# Autodesk Inventor assembly: hph_002
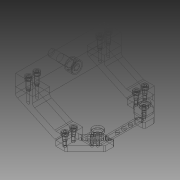
[picture p0: Inventor's stored thumbnail of the model, 180x180]
Saved by Autodesk Inventor 2014 (Build 180170000, 170)
## iProperties
Created: 2014-03-27
Part Number: hph_002
Document SubType Name: Assembly
Designer: stephenholtz
Author: stephenholtz
## Documents named in this file (11)
- C:\Users\stephenholtz\Dropbox\grad_school_docs\sabatini_lab_rotation\headpost_design\hph_001_full.iam
- C:\Users\stephenholtz\Dropbox\grad_school_docs\sabatini_lab_rotation\headpost_design\hph_C_001.ipt
- C:\Users\stephenholtz\Dropbox\grad_school_docs\sabatini_lab_rotation\headpost_design\hph_B_001.ipt
- C:\Users\stephenholtz\Dropbox\grad_school_docs\sabatini_lab_rotation\headpost_design\hph_A_001_left.ipt
- C:\Users\stephenholtz\Dropbox\grad_school_docs\sabatini_lab_rotation\headpost_design\hph_A_001_right.ipt
- C:\Users\stephenholtz\Dropbox\grad_school_docs\sabatini_lab_rotation\headpost_design\hph_D_001.ipt
- C:\Users\stephenholtz\Dropbox\grad_school_docs\sabatini_lab_rotation\headpost_design\hp_thick_001.ipt
- C:\Users\stephenholtz\Dropbox\grad_school_docs\sabatini_lab_rotation\headpost_design\standard_parts\4_-_40_hex_cap_screw.ipt
- C:\Users\stephenholtz\Dropbox\grad_school_docs\sabatini_lab_rotation\headpost_design\standard_parts\4_-_40_set_screw.ipt
- C:\Users\stephenholtz\Dropbox\grad_school_docs\sabatini_lab_rotation\headpost_design\standard_parts\wide_dia_knurled_shoulder_screw.ipt
- C:\Users\stephenholtz\Dropbox\grad_school_docs\sabatini_lab_rotation\headpost_design\standard_parts\1_4_-_20_hex_cap_screw.ipt
## Components (21 placed, 10 different names)
1. hph_C_001:1 — Mate:1, Mate:2, Mate:3, Mate:4, Flush:1, Flush:2, Rotational:1, Rotational:2, Rotational:3, Rotational:4, Rotational:5
2. hph_B_001:1 — Mate:1, Mate:3, Flush:1, Insert:1, Flush:3
3. hph_B_001:2 — Mate:2, Mate:4, Flush:2, Insert:2, Flush:4, Rotational:6, Rotational:7
4. hph_A_001_left:1 — Insert:2, Flush:4, Tangent:3, Tangent:4, Mate:5, Cylindrical:5, Cylindrical:6, Mate:7
5. hph_A_001_right:1 — Insert:1, Flush:3, Cylindrical:1, Cylindrical:2, Tangent:1, Tangent:2, Mate:6, Cylindrical:3, Cylindrical:4
6. hph_D_001:1 — Tangent:1, Tangent:2, Mate:6
7. hph_D_001:2 — Tangent:3, Tangent:4, Mate:5
8. hp_thick_001:1 — Mate:7
9. 4_-_40_hex_cap_screw:1 — Rotational:4
10. 4_-_40_hex_cap_screw:2 — Rotational:3
11. 4_-_40_hex_cap_screw:3 — Rotational:2
12. 4_-_40_hex_cap_screw:4 — Rotational:1
13. 4_-_40_hex_cap_screw:5 — Rotational:7
14. 4_-_40_hex_cap_screw:6 — Rotational:6
15. 4_-_40_hex_cap_screw:7 — Cylindrical:2
16. 4_-_40_hex_cap_screw:8 — Cylindrical:1
17. 4_-_40_set_screw:1 — Cylindrical:6
18. 4_-_40_set_screw:2 — Cylindrical:3
19. wide_dia_knurled_shoulder_screw:1 — Cylindrical:5
20. wide_dia_knurled_shoulder_screw:2 — Cylindrical:4
21. 1_4_-_20_hex_cap_screw:1 — Rotational:5
## Relationships (30: Mate 7, RevoluteJoint 7, CylindricalJoint 6, Flush 4, Tangent 4, Insert 2)
- Mate:1: hph_C_001:1 ↔ hph_B_001:1
- Mate:2: hph_C_001:1 ↔ hph_B_001:2
- Mate:3: hph_C_001:1 ↔ hph_B_001:1
- Mate:4: hph_C_001:1 ↔ hph_B_001:2
- Flush:1: hph_C_001:1 ↔ hph_B_001:1
- Flush:2: hph_C_001:1 ↔ hph_B_001:2
- Insert:1: hph_B_001:1 ↔ hph_A_001_right:1
- Flush:3: hph_B_001:1 ↔ hph_A_001_right:1
- Insert:2: hph_B_001:2 ↔ hph_A_001_left:1
- Flush:4: hph_B_001:2 ↔ hph_A_001_left:1
- Cylindrical:1: hph_A_001_right:1 ↔ 4_-_40_hex_cap_screw:8
- Cylindrical:2: hph_A_001_right:1 ↔ 4_-_40_hex_cap_screw:7
- Rotational:1 [RevoluteJoint]: hph_C_001:1 ↔ 4_-_40_hex_cap_screw:4
- Rotational:2 [RevoluteJoint]: hph_C_001:1 ↔ 4_-_40_hex_cap_screw:3
- Rotational:3 [RevoluteJoint]: hph_C_001:1 ↔ 4_-_40_hex_cap_screw:2
- Rotational:4 [RevoluteJoint]: hph_C_001:1 ↔ 4_-_40_hex_cap_screw:1
- Rotational:5 [RevoluteJoint]: hph_C_001:1 ↔ 1_4_-_20_hex_cap_screw:1
- Rotational:6 [RevoluteJoint]: hph_B_001:2 ↔ 4_-_40_hex_cap_screw:6
- Rotational:7 [RevoluteJoint]: hph_B_001:2 ↔ 4_-_40_hex_cap_screw:5
- Tangent:1: hph_A_001_right:1 ↔ hph_D_001:1
- Tangent:2: hph_A_001_right:1 ↔ hph_D_001:1
- Tangent:3: hph_A_001_left:1 ↔ hph_D_001:2
- Tangent:4: hph_A_001_left:1 ↔ hph_D_001:2
- Mate:5: hph_A_001_left:1 ↔ hph_D_001:2
- Mate:6: hph_A_001_right:1 ↔ hph_D_001:1
- Cylindrical:3: hph_A_001_right:1 ↔ 4_-_40_set_screw:2
- Cylindrical:4: hph_A_001_right:1 ↔ wide_dia_knurled_shoulder_screw:2
- Cylindrical:5: hph_A_001_left:1 ↔ wide_dia_knurled_shoulder_screw:1
- Cylindrical:6: hph_A_001_left:1 ↔ 4_-_40_set_screw:1
- Mate:7: hph_A_001_left:1 ↔ hp_thick_001:1
